# Autodesk Inventor assembly: step_66527
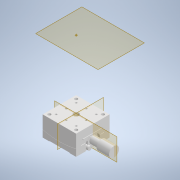
[picture p0: Inventor's stored thumbnail of the model, 180x180]
Saved by Autodesk Inventor 2022 (Build 260153000, 153)
## iProperties
Created: 2010-09-03
Part Number: step_66527
Description: STEP AP203
Document SubType Name: Assembly
Designer: gnzak
Sending System: SolidWorks 2007
Preprocessor: SwSTEP 2.0
Title: 66527.STEP
Comments: Radius: 3.22835 in or 82 mm
Revision Number: ANY
## Documents named in this file (2)
- C:\Users\gnzak\OneDrive\Documents\vr-frame-l7.033\Parts\Edmund Optics 66-527\step_66527.iam
- C:\Users\gnzak\OneDrive\Documents\vr-frame-l7.033\Parts\Edmund Optics 66-527\66527_ÃÞÌ«ÙÄ.ipt
## Components (1 placed, 1 different names)
1. 66527_ÃÞÌ«ÙÄ_1 — Flush:1, Flush:2, Flush:3, Flush:4, Flush:5
## Relationships (10: Flush 5, Mate 3, Symmetry 2)
- Flush:1 (82 mm): 66527_ÃÞÌ«ÙÄ_1
- Flush:2: 66527_ÃÞÌ«ÙÄ_1
- Flush:3: 66527_ÃÞÌ«ÙÄ_1
- Flush:4: 66527_ÃÞÌ«ÙÄ_1
- Flush:5: 66527_ÃÞÌ«ÙÄ_1
- Symmetry:1
- Symmetry:2
- Mate:1
- Mate:2
- Mate:3
